# Autodesk Inventor assembly: Клапан0
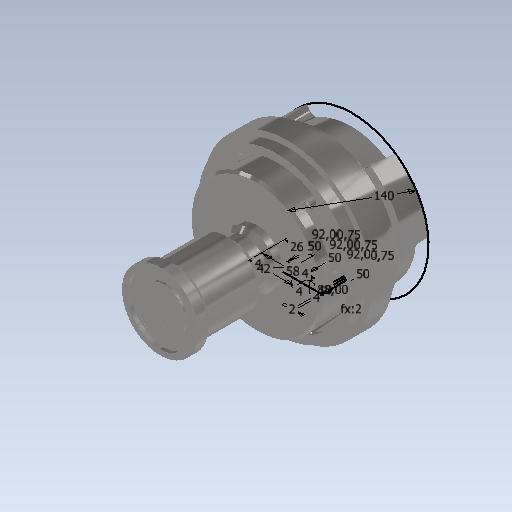
[picture p0: Inventor's stored thumbnail of the model, 512x512]
Saved by Autodesk Inventor 2021 (Build 250183000, 183)
## iProperties
Created: 2020-12-19
Part Number: Клапан0
Document SubType Name: Assembly
Designer: Тимоха
Author: Тимоха
## Documents named in this file (11)
- C:\Users\Тимоха\Desktop\КР Компрессор\compressor\Клапан0.iam
- C:\Users\Тимоха\Desktop\КР Компрессор\compressor\Ограничитель.ipt
- C:\Users\Тимоха\Desktop\КР Компрессор\compressor\Пластина.ipt
- C:\Users\Тимоха\Desktop\КР Компрессор\compressor\Седло.ipt
- C:\Users\Тимоха\Desktop\КР Компрессор\compressor\Для регулировки 1.ipt
- C:\Users\Тимоха\Desktop\КР Компрессор\compressor\Для регулировки 2.ipt
- C:\Users\Тимоха\Documents\Inventor\Content Center Files\R2021\ru-RU\GOST 5918-73 (2)\Гайка 2 M24-6H ГОСТ 5918-73.ipt
- C:\Users\Тимоха\Documents\Inventor\Content Center Files\R2021\ru-RU\Stud GOST 22038-76\Шпилька M24-6g×110 ГОСТ 22038-76.ipt
- C:\Users\Тимоха\Desktop\КР Компрессор\compressor\Вилка.ipt
- C:\Users\Тимоха\Desktop\КР Компрессор\compressor\Для регулировки 3.ipt
- C:\Users\Тимоха\Desktop\КР Компрессор\compressor\Для регулировки 4.ipt
## Components (10 placed, 10 different names)
1. Ограничитель:1 — Жесткий:1
2. Пластина:1 — Жесткий:2, Жесткий:6
3. Седло:1 — Жесткий:1, Жесткий:2, Жесткий:3, Жесткий:7
4. Для регулировки 1:2 — Жесткий:3, Жесткий:4
5. Для регулировки 2:1 — Жесткий:4, Жесткий:5
6. Гайка 2 ГОСТ 5918-73 M24:1 — Жесткий:5
7. Шпилька ГОСТ 22038-76 M24-6g×110:1 — Жесткий:6
8. Вилка:1 — Жесткий:7, Жесткий:8
9. Для регулировки 3:1 — Жесткий:8, Жесткий:9
10. Для регулировки 4:1 — Жесткий:9
## Relationships (9: WeldJoint 9)
- Жесткий:1 [WeldJoint]: Ограничитель:1 ↔ Седло:1
- Жесткий:2 [WeldJoint]: Пластина:1 ↔ Седло:1
- Жесткий:3 [WeldJoint]: Седло:1 ↔ Для регулировки 1:2
- Жесткий:4 [WeldJoint]: Для регулировки 1:2 ↔ Для регулировки 2:1
- Жесткий:5 [WeldJoint]: Для регулировки 2:1 ↔ Гайка 2 ГОСТ 5918-73 M24:1
- Жесткий:6 [WeldJoint]: Пластина:1 ↔ Шпилька ГОСТ 22038-76 M24-6g×110:1
- Жесткий:7 [WeldJoint] (19 mm): Седло:1 ↔ Вилка:1
- Жесткий:8 [WeldJoint]: Вилка:1 ↔ Для регулировки 3:1
- Жесткий:9 [WeldJoint]: Для регулировки 3:1 ↔ Для регулировки 4:1
